# Autodesk Inventor assembly: elevator
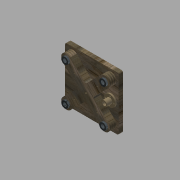
[picture p0: Inventor's stored thumbnail of the model, 180x180]
Saved by Autodesk Inventor 2019 (Build 230136000, 136)
## iProperties
Created: 2021-11-01
Part Number: elevator
Document SubType Name: Assembly
Designer: Mohamed
Author: Mohamed
## Documents named in this file (6)
- F:\Semester 7\Design of mechatronics 1\SSCARA Robot\elevator.iam
- F:\Semester 7\Design of mechatronics 1\SSCARA Robot\E_base1.ipt
- F:\Semester 7\Design of mechatronics 1\SSCARA Robot\e_guid nut.ipt
- F:\Semester 7\Design of mechatronics 1\SSCARA Robot\E_base2.ipt
- F:\Semester 7\Design of mechatronics 1\SSCARA Robot\e_linear bearing 10mm.ipt
- F:\Semester 7\Design of mechatronics 1\SSCARA Robot\e_support 1.ipt
## Components (10 placed, 5 different names)
1. E_base1:1 — Mate:1, Mate:2, Mate:3, Mate:4, Mate:5, Mate:6, Mate:7, Mate:8, Mate:10, Mate:17
2. e_guid nut:1 — Mate:1, Mate:2
3. E_base2:1 — Mate:3, Mate:4, Mate:5, Mate:6, Mate:9, Mate:11, Mate:12, Mate:13, Mate:14
4. e_linear bearing 10mm:1 — Mate:8, Mate:13
5. e_linear bearing 10mm:2 — Mate:9, Mate:11
6. e_linear bearing 10mm:3 — Mate:10, Mate:12, Mate:15, Mate:18, Mate:22
7. e_linear bearing 10mm:4 — Mate:7, Mate:14, Mate:16, Mate:19, Mate:21
8. e_support 1:1 — Mate:15, Mate:16, Mate:17, Mate:20
9. e_support 1:2 — Mate:18, Mate:19, Mate:20, Mate:23
10. e_support 1:3 — Mate:21, Mate:22, Mate:23
## Relationships (23: Mate 23)
- Mate:1: E_base1:1 ↔ e_guid nut:1
- Mate:2: E_base1:1 ↔ e_guid nut:1
- Mate:3: E_base1:1 ↔ E_base2:1
- Mate:4: E_base1:1 ↔ E_base2:1
- Mate:5: E_base1:1 ↔ E_base2:1
- Mate:6: E_base1:1 ↔ E_base2:1
- Mate:7: E_base1:1 ↔ e_linear bearing 10mm:4
- Mate:8: E_base1:1 ↔ e_linear bearing 10mm:1
- Mate:9: E_base2:1 ↔ e_linear bearing 10mm:2
- Mate:10: E_base1:1 ↔ e_linear bearing 10mm:3
- Mate:11: E_base2:1 ↔ e_linear bearing 10mm:2
- Mate:12: E_base2:1 ↔ e_linear bearing 10mm:3
- Mate:13: E_base2:1 ↔ e_linear bearing 10mm:1
- Mate:14: E_base2:1 ↔ e_linear bearing 10mm:4
- Mate:15: e_linear bearing 10mm:3 ↔ e_support 1:1
- Mate:16: e_linear bearing 10mm:4 ↔ e_support 1:1
- Mate:17: E_base1:1 ↔ e_support 1:1
- Mate:18: e_linear bearing 10mm:3 ↔ e_support 1:2
- Mate:19: e_linear bearing 10mm:4 ↔ e_support 1:2
- Mate:20: e_support 1:1 ↔ e_support 1:2
- Mate:21: e_linear bearing 10mm:4 ↔ e_support 1:3
- Mate:22: e_linear bearing 10mm:3 ↔ e_support 1:3
- Mate:23: e_support 1:2 ↔ e_support 1:3
